# Autodesk Inventor assembly: module_pms7003
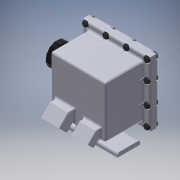
[picture p0: Inventor's stored thumbnail of the model, 180x180]
Saved by Autodesk Inventor 2018 (Build 220112000, 112)
## iProperties
Created: 2019-04-22
Part Number: module_pms7003
Document SubType Name: Assembly
Designer: ZEUSLAP
Author: ZEUSLAP
## Documents named in this file (9)
- C:\Users\ZEUSLAP\Desktop\comparative-air-pollution-sensor\models\module_pms7003\module_pms7003.iam
- C:\Users\ZEUSLAP\Desktop\comparative-air-pollution-sensor\models\module_pms7003\parts\plantower-pms7003-laser-dust-sensor\pms7003.iam
- C:\Users\ZEUSLAP\Desktop\comparative-air-pollution-sensor\models\module_ppd42\parts\SP16 waterproof connector\SP16-4P, female, back nut type.iam
- C:\Users\ZEUSLAP\Desktop\comparative-air-pollution-sensor\models\module_pms7003\parts\SP16 waterproof connector\parts\nut.ipt
- C:\Users\ZEUSLAP\Desktop\comparative-air-pollution-sensor\models\module_pms7003\parts\SP16 waterproof connector\parts\rubber_washer.ipt
- C:\Users\ZEUSLAP\Desktop\comparative-air-pollution-sensor\models\module_pms7003\enclosure\enclosure.ipt
- C:\Users\ZEUSLAP\Desktop\comparative-air-pollution-sensor\models\module_pms7003\enclosure\lid.ipt
- C:\Users\ZEUSLAP\Documents\Inventor\Content Center Files\R2018\en-US\ISO 7045  H\ISO 7045 - M3 x 8 - 4.8 - H - ISO.ipt
- C:\Users\ZEUSLAP\Documents\Inventor\Content Center Files\R2018\en-US\ISO 4032(2)\ISO 4032 - M3 - ISO.ipt
## Components (30 placed, 8 different names)
1. pms7003:1 [sub-assembly] — Mate:3, Mate:4, Mate:5
2. SP16-4P, female, back nut type:1 [sub-assembly] — Mate:8, Mate:9, Mate:11
3. nut:1 — Mate:10, Mate:11
4. rubber_washer:1 — Mate:6, Mate:7, Mate:8
5. enclosure:1 — Mate:3, Mate:4, Mate:5, Mate:6, Mate:7, Mate:9, Mate:10, Mate:12, Mate:13, Mate:14, Insert:1, Insert:3, Insert:4, Insert:5, Insert:6, Insert:7, Insert:8, Insert:9, Insert:10, Insert:11, Insert:12, Mate:40, Angle:13
6. lid:1 — Mate:12, Mate:13, Mate:14, Mate:16, Mate:20, Mate:22, Mate:24, Mate:26, Mate:28, Mate:30, Mate:32, Mate:34, Mate:36, Mate:38, Angle:1, Angle:3, Angle:4, Angle:5, Angle:6, Angle:7, Angle:8, Angle:9, Angle:10, Angle:11, Angle:12, Insert:13
7. ISO 7045 H M3 x 8 - 4.8 - H:1 — Insert:1, Mate:37
8. ISO 7045 H M3 x 8 - 4.8 - H:3 — Insert:3, Mate:19
9. ISO 7045 H M3 x 8 - 4.8 - H:4 — Insert:4, Mate:21
10. ISO 7045 H M3 x 8 - 4.8 - H:5 — Insert:5, Mate:23
11. ISO 7045 H M3 x 8 - 4.8 - H:6 — Insert:6, Mate:33
12. ISO 7045 H M3 x 8 - 4.8 - H:7 — Insert:7, Mate:35
13. ISO 7045 H M3 x 8 - 4.8 - H:8 — Insert:8, Mate:31
14. ISO 7045 H M3 x 8 - 4.8 - H:9 — Insert:9, Mate:29
15. ISO 7045 H M3 x 8 - 4.8 - H:10 — Insert:10, Mate:25
16. ISO 7045 H M3 x 8 - 4.8 - H:11 — Insert:11, Mate:15
17. ISO 7045 H M3 x 8 - 4.8 - H:12 — Insert:12, Mate:27
18. ISO 4032 M3:1 — Mate:15, Mate:16, Angle:1
19. ISO 4032 M3:3 — Mate:19, Mate:20, Angle:3
20. ISO 4032 M3:4 — Mate:21, Mate:22, Angle:4
21. ISO 4032 M3:5 — Mate:23, Mate:24, Angle:5
22. ISO 4032 M3:6 — Mate:25, Mate:26, Angle:6
23. ISO 4032 M3:7 — Mate:27, Mate:28, Angle:7
24. ISO 4032 M3:8 — Mate:29, Mate:30, Angle:8
25. ISO 4032 M3:9 — Mate:31, Mate:32, Angle:9
26. ISO 4032 M3:10 — Mate:33, Mate:34, Angle:10
27. ISO 4032 M3:11 — Mate:35, Mate:36, Angle:11
28. ISO 4032 M3:12 — Mate:37, Mate:38, Angle:12
29. ISO 7045 H M3 x 8 - 4.8 - H:13 — Insert:13, Mate:39
30. ISO 4032 M3:13 — Mate:39, Mate:40, Angle:13
## Relationships (60: Mate 36, Insert 12, Angle 12)
- Mate:3: pms7003:1 ↔ enclosure:1
- Mate:4: pms7003:1 ↔ enclosure:1
- Mate:5: pms7003:1 ↔ enclosure:1
- Mate:6: rubber_washer:1 ↔ enclosure:1
- Mate:7: rubber_washer:1 ↔ enclosure:1
- Mate:8: SP16-4P, female, back nut type:1 ↔ rubber_washer:1
- Mate:9: SP16-4P, female, back nut type:1 ↔ enclosure:1
- Mate:10: nut:1 ↔ enclosure:1
- Mate:11: SP16-4P, female, back nut type:1 ↔ nut:1
- Mate:12: enclosure:1 ↔ lid:1
- Mate:13: enclosure:1 ↔ lid:1
- Mate:14: enclosure:1 ↔ lid:1
- Insert:1: enclosure:1 ↔ ISO 7045 H M3 x 8 - 4.8 - H:1
- Insert:3: enclosure:1 ↔ ISO 7045 H M3 x 8 - 4.8 - H:3
- Insert:4: enclosure:1 ↔ ISO 7045 H M3 x 8 - 4.8 - H:4
- Insert:5: enclosure:1 ↔ ISO 7045 H M3 x 8 - 4.8 - H:5
- Insert:6: enclosure:1 ↔ ISO 7045 H M3 x 8 - 4.8 - H:6
- Insert:7: enclosure:1 ↔ ISO 7045 H M3 x 8 - 4.8 - H:7
- Insert:8: enclosure:1 ↔ ISO 7045 H M3 x 8 - 4.8 - H:8
- Insert:9: enclosure:1 ↔ ISO 7045 H M3 x 8 - 4.8 - H:9
- Insert:10: enclosure:1 ↔ ISO 7045 H M3 x 8 - 4.8 - H:10
- Insert:11: enclosure:1 ↔ ISO 7045 H M3 x 8 - 4.8 - H:11
- Insert:12: enclosure:1 ↔ ISO 7045 H M3 x 8 - 4.8 - H:12
- Mate:15: ISO 7045 H M3 x 8 - 4.8 - H:11 ↔ ISO 4032 M3:1
- Mate:16: lid:1 ↔ ISO 4032 M3:1
- Mate:19: ISO 7045 H M3 x 8 - 4.8 - H:3 ↔ ISO 4032 M3:3
- Mate:20: lid:1 ↔ ISO 4032 M3:3
- Mate:21: ISO 7045 H M3 x 8 - 4.8 - H:4 ↔ ISO 4032 M3:4
- Mate:22: lid:1 ↔ ISO 4032 M3:4
- Mate:23: ISO 7045 H M3 x 8 - 4.8 - H:5 ↔ ISO 4032 M3:5
- Mate:24: lid:1 ↔ ISO 4032 M3:5
- Mate:25: ISO 7045 H M3 x 8 - 4.8 - H:10 ↔ ISO 4032 M3:6
- Mate:26: lid:1 ↔ ISO 4032 M3:6
- Mate:27: ISO 7045 H M3 x 8 - 4.8 - H:12 ↔ ISO 4032 M3:7
- Mate:28: lid:1 ↔ ISO 4032 M3:7
- Mate:29: ISO 7045 H M3 x 8 - 4.8 - H:9 ↔ ISO 4032 M3:8
- Mate:30: lid:1 ↔ ISO 4032 M3:8
- Mate:31: ISO 7045 H M3 x 8 - 4.8 - H:8 ↔ ISO 4032 M3:9
- Mate:32: lid:1 ↔ ISO 4032 M3:9
- Mate:33: ISO 7045 H M3 x 8 - 4.8 - H:6 ↔ ISO 4032 M3:10
- Mate:34: lid:1 ↔ ISO 4032 M3:10
- Mate:35: ISO 7045 H M3 x 8 - 4.8 - H:7 ↔ ISO 4032 M3:11
- Mate:36: lid:1 ↔ ISO 4032 M3:11
- Mate:37: ISO 7045 H M3 x 8 - 4.8 - H:1 ↔ ISO 4032 M3:12
- Mate:38: lid:1 ↔ ISO 4032 M3:12
- Angle:1 (90 deg): lid:1 ↔ ISO 4032 M3:1
- Angle:3 (90 deg): lid:1 ↔ ISO 4032 M3:3
- Angle:4 (90 deg): lid:1 ↔ ISO 4032 M3:4
- Angle:5 (90 deg): lid:1 ↔ ISO 4032 M3:5
- Angle:6 (90 deg): lid:1 ↔ ISO 4032 M3:6
- Angle:7 (90 deg): lid:1 ↔ ISO 4032 M3:7
- Angle:8 (90 deg): lid:1 ↔ ISO 4032 M3:8
- Angle:9 (90 deg): lid:1 ↔ ISO 4032 M3:9
- Angle:10 (90 deg): lid:1 ↔ ISO 4032 M3:10
- Angle:11 (90 deg): lid:1 ↔ ISO 4032 M3:11
- Angle:12 (90 deg): lid:1 ↔ ISO 4032 M3:12
- Insert:13: lid:1 ↔ ISO 7045 H M3 x 8 - 4.8 - H:13
- Mate:39: ISO 7045 H M3 x 8 - 4.8 - H:13 ↔ ISO 4032 M3:13
- Mate:40: enclosure:1 ↔ ISO 4032 M3:13
- Angle:13 (90 deg): enclosure:1 ↔ ISO 4032 M3:13
